# Autodesk Inventor assembly: Sonar-Box
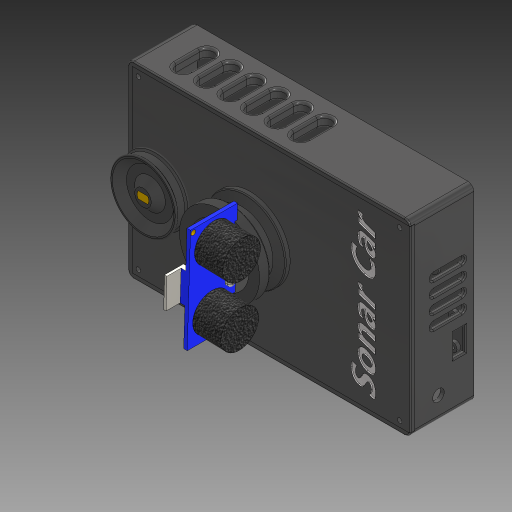
[picture p0: Inventor's stored thumbnail of the model, 512x512]
Saved by Autodesk Inventor 2023 (Build 270158000, 158)
## iProperties
Created: 2024-02-02
Part Number: Sonar-Box
Document SubType Name: Assembly
Designer: matej
Author: matej
## Documents named in this file (9)
- C:\Users\matej\Documents\GitHub\Sonar-Car\models\Sonar\Sonar-Box.iam
- C:\Users\matej\Documents\GitHub\Sonar-Car\models\Sonar\box.ipt
- C:\Users\matej\Documents\GitHub\Sonar-Car\models\Sonar\box-top.ipt
- C:\Users\matej\Documents\GitHub\Sonar-Car\models\Sonar\OtocnaKontaktniPruchodka.ipt
- C:\Users\matej\Documents\GitHub\Sonar-Car\models\Sonar\StepperMotor.ipt
- C:\Users\matej\Documents\GitHub\Sonar-Car\models\Sonar\rub-ring.ipt
- C:\Users\matej\Documents\GitHub\Sonar-Car\models\Sonar\support-ring.ipt
- C:\Users\matej\Documents\GitHub\Sonar-Car\models\Sonar\sonar.ipt
- C:\Users\matej\Documents\GitHub\Sonar-Car\models\Sonar\UltraZvuk.ipt
## Components (8 placed, 8 different names)
1. box:1 — Tuhé:2, Posuvné:1
2. box-top:1 — Tuhé:1, Posuvné:1
3. OtocnaKontaktniPruchodka:1 — Tuhé:1, Rotační:1, Vložit:1
4. StepperMotor:1 — Tuhé:2, Proti sobě:1, Proti sobě:3, Proti sobě:4
5. rub-ring:1 — Proti sobě:1, Proti sobě:3, Proti sobě:4
6. support-ring:1 — Vložit:1
7. sonar:1 — Rotační:1, Proti sobě:6, Proti sobě:7
8. UltraZvuk:1 — Proti sobě:6, Proti sobě:7
## Relationships (10: Mate 5, WeldJoint 2, RevoluteJoint 1, Insert 1, TranslationJoint 1)
- Tuhé:1 [WeldJoint]: box-top:1 ↔ OtocnaKontaktniPruchodka:1
- Tuhé:2 [WeldJoint]: box:1 ↔ StepperMotor:1
- Proti sobě:1 [Mate]: StepperMotor:1 ↔ rub-ring:1
- Proti sobě:3 [Mate]: StepperMotor:1 ↔ rub-ring:1
- Proti sobě:4 [Mate]: StepperMotor:1 ↔ rub-ring:1
- Rotační:1 [RevoluteJoint]: OtocnaKontaktniPruchodka:1 ↔ sonar:1
- Proti sobě:6 [Mate]: sonar:1 ↔ UltraZvuk:1
- Vložit:1 [Insert]: OtocnaKontaktniPruchodka:1 ↔ support-ring:1
- Posuvné:1 [TranslationJoint]: box:1 ↔ box-top:1
- Proti sobě:7 [Mate]: sonar:1 ↔ UltraZvuk:1
